# Autodesk Inventor assembly: knee_fin1
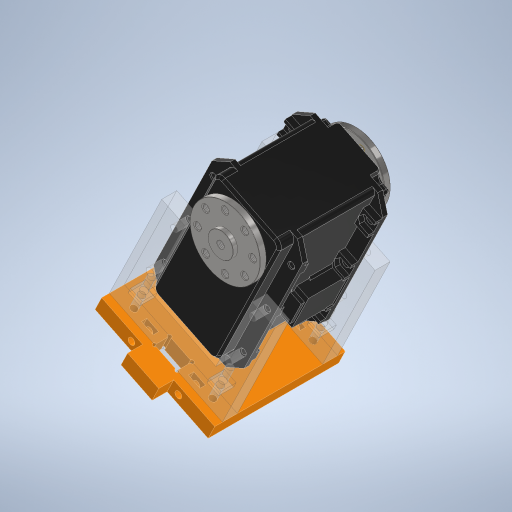
[picture p0: Inventor's stored thumbnail of the model, 512x512]
Saved by Autodesk Inventor 2024 (Build 280153000, 153)
## iProperties
Created: 2024-09-16
Part Number: knee_fin1
Document SubType Name: Assembly
Designer: jmha0
Author: jmha0
## Documents named in this file (6)
- C:\Users\jmha0\OneDrive\바탕 화면\19th_intern_hjm_fight_robot\부품\Lower_Body\knee_w_motor\knee_fin1.iam
- C:\Users\jmha0\OneDrive\바탕 화면\19th_intern_hjm_fight_robot\부품\hardware\ROBOTIS(Inventor 2024 ver.)\다이나믹셀\MX-106T+idle.ipt.iam
- C:\Users\jmha0\OneDrive\바탕 화면\19th_intern_hjm_fight_robot\부품\hardware\ROBOTIS(Inventor 2024 ver.)\혼\64-106Horn.ipt
- C:\Users\jmha0\OneDrive\바탕 화면\19th_intern_hjm_fight_robot\부품\Lower_Body\knee_w_motor\frame_knee_to_bridge.ipt
- C:\Users\jmha0\OneDrive\바탕 화면\19th_intern_hjm_fight_robot\부품\Lower_Body\knee_w_motor\bridge1.ipt
- MX-106T+idle.ipt
## Components (5 placed, 4 different names)
1. MX-106T+idle.ipt:1 [sub-assembly] — 삽입:7, 삽입:8
2. 64-106Horn:1
3. frame_knee_to_bridge:1
4. bridge1:1 — 삽입:9, 삽입:10
5. frame_knee_to_bridge:2 — 삽입:7, 삽입:8, 삽입:9, 삽입:10
## Relationships (10: Insert 10)
- [Insert] (0.1 mm): MX-106T+idle.ipt:1 ↔ 64-106Horn:1
- [Insert]: MX-106T+idle.ipt:1 ↔ frame_knee_to_bridge:1
- [Insert]: MX-106T+idle.ipt:1 ↔ frame_knee_to_bridge:1
- [Insert]: MX-106T+idle.ipt:1 ↔ frame_knee_to_bridge:1
- [Insert]: frame_knee_to_bridge:1 ↔ bridge1:1
- [Insert]: frame_knee_to_bridge:1 ↔ bridge1:1
- 삽입:7 [Insert]: MX-106T+idle.ipt:1 ↔ frame_knee_to_bridge:2
- 삽입:8 [Insert]: MX-106T+idle.ipt:1 ↔ frame_knee_to_bridge:2
- 삽입:9 [Insert]: bridge1:1 ↔ frame_knee_to_bridge:2
- 삽입:10 [Insert]: bridge1:1 ↔ frame_knee_to_bridge:2
